# Autodesk Inventor assembly: dron_all
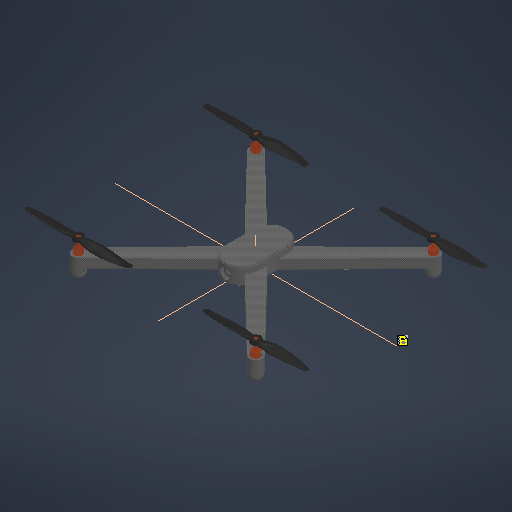
[picture p0: Inventor's stored thumbnail of the model, 512x512]
Saved by Autodesk Inventor 2026 (Build 300175050, 175E)
## iProperties
Created: 2026-03-25
Part Number: dron_all
Document SubType Name: Assembly
Designer: josef
Mass: 2408.89 g
Surface Area: 2519.22 cm^2
Volume: 1391.75 cm^3
Density: 1.73083 g/cm^3
Author: josef
## Documents named in this file (5)
- C:\Users\josef\OneDrive\Dokumenty\msc_adams\dron_all.iam
- C:\Users\josef\OneDrive\Dokumenty\msc_adams\dronek.ipt
- C:\Users\josef\Downloads\prop-ccw10x4-5-1.snapshot.2\PropellerCCW10x4,5 v6\PropellerCCW10x4,5 v6\PropellerCCW10x4,5.ipt
- C:\Users\josef\OneDrive\Dokumenty\msc_adams\motor.ipt
- C:\Users\josef\OneDrive\Dokumenty\msc_adams\pcb_aproximace.ipt
## Components (10 placed, 4 different names)
1. dronek:1 — Mate:1, Flush:3, Mate:3, Mate:4, Mate:5, Mate:6, Mate:7, Mate:8, Mate:9, Mate:10, Mate:11, Mate:20, Mate:22, Flush:5, Flush:6
2. PropellerCCW10x4,5:1 — Mate:13, Mate:18, Mate:25
3. PropellerCCW10x4,5:2 — Mate:24, Flush:4, Mate:26
4. PropellerCCW10x4,5:3 — Mate:14, Mate:16, Mate:27
5. PropellerCCW10x4,5:4 — Mate:17, Mate:23, Mate:28
6. motor:1 — Mate:6, Mate:9, Mate:13, Mate:18
7. motor:2 — Mate:5, Mate:11, Mate:24, Flush:4
8. motor:3 — Mate:4, Mate:8, Mate:14, Mate:16
9. motor:4 — Mate:7, Mate:10, Mate:17, Mate:23
10. pcb_aproximace:1 — Mate:20, Mate:22
## Relationships (27: Mate 23, Flush 4)
- Mate:1: dronek:1
- Flush:3: dronek:1
- Mate:3: dronek:1
- Mate:4: dronek:1 ↔ motor:3
- Mate:5: dronek:1 ↔ motor:2
- Mate:6: dronek:1 ↔ motor:1
- Mate:7: dronek:1 ↔ motor:4
- Mate:8: dronek:1 ↔ motor:3
- Mate:9: dronek:1 ↔ motor:1
- Mate:10: dronek:1 ↔ motor:4
- Mate:11: dronek:1 ↔ motor:2
- Mate:13: PropellerCCW10x4,5:1 ↔ motor:1
- Mate:14: PropellerCCW10x4,5:3 ↔ motor:3
- Mate:16: PropellerCCW10x4,5:3 ↔ motor:3
- Mate:17: PropellerCCW10x4,5:4 ↔ motor:4
- Mate:18: PropellerCCW10x4,5:1 ↔ motor:1
- Mate:20: dronek:1 ↔ pcb_aproximace:1
- Mate:22: dronek:1 ↔ pcb_aproximace:1
- Mate:23: PropellerCCW10x4,5:4 ↔ motor:4
- Mate:24: PropellerCCW10x4,5:2 ↔ motor:2
- Flush:4: PropellerCCW10x4,5:2 ↔ motor:2
- Flush:5 (212.132 mm): dronek:1
- Mate:25: PropellerCCW10x4,5:1
- Mate:26: PropellerCCW10x4,5:2
- Flush:6 (-212.132 mm): dronek:1
- Mate:27: PropellerCCW10x4,5:3
- Mate:28: PropellerCCW10x4,5:4
